# Autodesk Inventor assembly: 3_left_leg_true_final
(part 3 of 3)
Size Designation: M3 x 6
Categories: <MemberInstance><Categories><Category DisplayName="Fasteners" InternalName="e4da775c-781d-43d5-af7c-5136215cf5a6" Mnemonic="FSTN"><Category DisplayName="Bolts" InternalName="536e6df0-f778-49ac-b2f2-25c71d2aa0b2" Mnemonic="SCRW"><CategoryParameter DisplayName="Nominal Diameter Designation" InternalName="03caf894-eafd-4c09-a035-916ac084b87b" Mnemonic="nomdiadesig"/><CategoryParameter DisplayName="Nominal Length" InternalName="238ecbaf-3e6c-45dd-aa95-4068c8e0fd02" Mnemonic="nomlen"/><CategoryParameter DisplayName="Thread Designation" InternalName="586d5e89-370a-4089-914f-0110033585c7" Mnemonic="thrdesign"/><CategoryParameter DisplayName="Thread Series Designation" InternalName="87c5849c-b3a5-4c3e-9c9b-2feecef9be86" Mnemonic="thrserdsgn"/><CategoryParameter DisplayName="Nominal Diameter" InternalName="8bbe3f8e-44cf-40a9-a251-3a6edc8168d6" Mnemonic="nomdia"/><CategoryParameter DisplayName="Thread Type" InternalName="b4bbb7bc-d6aa-4c9f-a9a9-4152b9f6fe49" Mnemonic="thrtype"/><CategoryParameter DisplayName="Thread Pitch" InternalName="bb82302e-82d8-4176-8fc1-c5d7bb17d5ad" Mnemonic="pitch1"/><CategoryParameter DisplayName="Threads per Unit" InternalName="bdc6e7d2-ffd0-4d9c-a173-16b95ebb912d" Mnemonic="thrperunit1"/><CategoryParameter DisplayName="Thread Class" InternalName="ebc0d23b-2cc6-4d2a-b376-d52aae53bab6" Mnemonic="thrclss"/><Category DisplayName="Round Head" InternalName="df3578aa-538f-4805-96a8-2439eb0c3cf7" Mnemonic="RNDSCRW"><CategoryParameter DisplayName="Grip Length" InternalName="2c6ace26-543b-4217-91c4-9cdf8c3ec6f1" Mnemonic="grplen"/><CategoryParameter DisplayName="Head Height" InternalName="2d152238-84fe-49ae-94c3-3fee884c292b" Mnemonic="headh"/><CategoryParameter DisplayName="Property Class" InternalName="85496db6-1567-48ed-b0d4-aa1f03366005" Mnemonic="propclss"/><CategoryParameter DisplayName="Thread Length" InternalName="a1e5edc5-4ca7-4847-8786-65b14d35af16" Mnemonic="thrlen"/><CategoryParameter DisplayName="Shank Diameter" InternalName="c22f1a48-b8d5-43ef-ac5e-546ba91c0bd6" Mnemonic="grpdia"/><CategoryParameter DisplayName="Head Diameter" InternalName="e71ee7a1-06fd-425c-ba3b-09769885677c" Mnemonic="headdia"/></Category></Category></Category><Category DisplayName="DataType" InternalName="23b78d0f-2648-40c6-8793-ca6db495c9e8" Mnemonic="DATATYPE"><CategoryParameter DisplayName="DisplayName" InternalName="05415f3d-3907-474b-a020-eb9d644f4cf3" Mnemonic="DISPLAYNAME"/><CategoryParameter DisplayName="Standard" InternalName="0c0a119c-1e12-4c84-803f-101930972f5e" Mnemonic="STANDARD"/><CategoryParameter DisplayName="Description" InternalName="13903e3d-64b1-4950-80da-f627842ea37f" Mnemonic="DESCRIPTION"/><CategoryParameter DisplayName="Designation" InternalName="2675968c-4ce5-49e0-a4f5-552d29089031" Mnemonic="DESIGNATION"/><CategoryParameter DisplayName="Default Row" InternalName="2af9ec52-faaa-4026-b378-f9fa4afca842" Mnemonic="DEFAULTROW"/><CategoryParameter DisplayName="Folder Name" InternalName="3f06958e-8713-4116-9be7-ed6184ecc97b" Mnemonic="FOLDERNAME"/><CategoryParameter DisplayName="Revision Guid" InternalName="45a75005-10b1-4dfc-8d6d-dfe629f0b93c" Mnemonic="REVISIONGUID"/><CategoryParameter DisplayName="FileName" InternalName="8b46a4cc-9585-4fed-90c3-899f57e09a73" Mnemonic="FILENAME"/><CategoryParameter DisplayName="StdsOrg" InternalName="8f5914e1-4693-403f-8ab5-d37768198c9d" Mnemonic="STDSORG"/><CategoryParameter DisplayName="Family Version" InternalName="914462f6-6e19-4b14-ba84-155b9680b1d0" Mnemonic="FAMILYREVISION"/><CategoryParameter DisplayName="Standard Revision" InternalName="91d5a463-65c2-4fde-b823-3b7fea5e8e17" Mnemonic="STANDARDREVISION"/><CategoryParameter DisplayName="Member Revision" InternalName="a65d44b9-392f-4f4f-857b-e4b3d54996fe" Mnemonic="MEMBERREVISION"/><CategoryParameter DisplayName="ClipFormat" InternalName="bc51e27b-3422-4e78-93ef-cec197ddf230" Mnemonic="CLIPFORMAT"/><CategoryParameter DisplayName="Manufacturer" InternalName="cd6c7a72-a28a-4e50-99a9-2c7f4e13e5ad" Mnemonic="MANUFACTURER"/><CategoryParameter DisplayName="InternalName" InternalName="cf1d0246-76d9-4b4a-8305-fa0409afb5c1" Mnemonic="INTERNALNAME"/><CategoryParameter DisplayName="IsMetric" InternalName="e2385c5b-1ea4-4823-96a8-8de651266ec3" Mnemonic="ISMETRIC"/><Category DisplayName="Part" InternalName="c0e0b642-3bcb-4cc8-9e80-f96d35c4afa4" Mnemonic="PART"><CategoryParameter DisplayName="Part Number" InternalName="016b6077-bfbe-49bd-92c9-d8d59c39c941" Mnemonic="PARTNUMBER"/><CategoryParameter DisplayName="Stock Number" InternalName="4dba7c1c-e26c-444e-836c-b08b433409a8" Mnemonic="STOCKNUMBER"/><CategoryParameter DisplayName="Material Key" InternalName="5c9a8adb-dd2b-4535-b97f-0a94a95fe41f" Mnemonic="MATERIALKEY"/><CategoryParameter DisplayName="Material" InternalName="818a152a-d3c3-49ca-80ee-df7d91421b8e" Mnemonic="MATERIAL"/></Category></Category><Category DisplayName="LegacyMap" InternalName="cd87c42b-3e48-431e-b5c0-1cbeb14dfe77" Mnemonic="LEGACYMAP"><CategoryParameter DisplayName="unique DA member ID" InternalName="0918ad47-427f-4fed-ae26-24c81c58f590" Mnemonic="DACOOKIE"/><CategoryParameter DisplayName="Merge11 ID" InternalName="0ee8fb18-e2ed-4f39-96f6-1f4b5f50aa71" Mnemonic="MERGE11"/><CategoryParameter DisplayName="unique CC member ID" InternalName="5193edd4-b2b0-4ab4-9d54-de900eee34e0" Mnemonic="CCCOOKIE"/><CategoryParameter DisplayName="Split ID" InternalName="72b5c83c-be7f-45c4-ae51-9160ea6deb26" Mnemonic="SPLIT"/><CategoryParameter DisplayName="MemberID" InternalName="8e5e0294-fc51-4c8f-b3d7-003dc5ed94f6" Mnemonic="MEMBERID"/><CategoryParameter DisplayName="CatalogName" InternalName="d99d1e27-aa94-4de2-af4c-c348882a6f4f" Mnemonic="CATALOGNAME"/><CategoryParameter DisplayName="FamilyNumber" InternalName="e705e1f4-09cb-413e-91f9-551b4188271e" Mnemonic="FAMILYNUMBER"/></Category></Categories><FamilyTemplate Id="si0145"><FamilyTemplateParameters><FamilyTemplateParameter ObjectType="kUserParameterObject" ValueType="xs:double" Id="1" ObjectReferenceKey="GUL"/><FamilyTemplateParameter ObjectType="kUserParameterObject" ValueType="xs:double" Id="2" ObjectReferenceKey="SPD"/><FamilyTemplateParameter ObjectType="kUserParameterObject" ValueType="xs:double" Id="3" ObjectReferenceKey="NLG"/><FamilyTemplateParameter ObjectType="kUserParameterObject" ValueType="xs:double" Id="4" ObjectReferenceKey="TPU"/><FamilyTemplateParameter ObjectType="kUserParameterObject" ValueType="xs:double" Id="5" ObjectReferenceKey="TOA"/><FamilyTemplateParameter ObjectType="kUserParameterObject" ValueType="xs:double" Id="6" ObjectReferenceKey="GD1"/><FamilyTemplateParameter ObjectType="kUserParameterObject" ValueType="xs:double" Id="7" ObjectReferenceKey="GEL"/><FamilyTemplateParameter ObjectType="kUserParameterObject" ValueType="xs:double" Id="8" ObjectReferenceKey="SW"/><FamilyTemplateParameter ObjectType="kUserParameterObject" ValueType="xs:double" Id="9" ObjectReferenceKey="THREADDIA"/><FamilyTemplateParameter ObjectType="kUserParameterObject" ValueType="xs:double" Id="10" ObjectReferenceKey="INTI"/><FamilyTemplateParameter ObjectType="kUserParameterObject" ValueType="xs:double" Id="11" ObjectReferenceKey="BDM"/><FamilyTemplateParameter ObjectType="kUserParameterObject" ValueType="xs:double" Id="12" ObjectReferenceKey="RR"/><FamilyTemplateParameter ObjectType="kUserParameterObject" ValueType="xs:double" Id="13" ObjectReferenceKey="KOH"/><FamilyTemplateParameter ObjectType="kUserParameterObject" ValueType="xs:double" Id="14" ObjectReferenceKey="PTC"/><FamilyTemplateParameter ObjectType="kUserParameterObject" ValueType="xs:double" Id="15" ObjectReferenceKey="KOD"/><FamilyTemplateParameter ObjectType="kUserParameterObject" ValueType="xs:double" Id="16" ObjectReferenceKey="NND"/><FamilyTemplateParameter ObjectType="kUserParameterObject" ValueType="xs:double" Id="17" ObjectReferenceKey="GD"/><FamilyTemplateParameter ObjectType="kUserParameterObject" ValueType="xs:double" Id="18" ObjectReferenceKey="GAL"/><FamilyTemplateParameter ObjectType="kUserParameterObject" ValueType="xs:double" Id="19" ObjectReferenceKey="KOH1"/><FamilyTemplateParameter ObjectType="kUserParameterObject" ValueType="xs:double" Id="20" ObjectReferenceKey="E0"/><FamilyTemplateParameter ObjectType="kUserParameterObject" ValueType="xs:double" Id="132" ObjectReferenceKey="R"/><FamilyTemplateParameter ObjectType="kPropertyObject" ValueType="xs:string" Id="100" ObjectReferenceKey="{32853F0F-3444-11d1-9E93-0060B03C1CA6}" SubObjectId="52"/><FamilyTemplateParameter ObjectType="kPropertyObject" ValueType="xs:string" Id="105" ObjectReferenceKey="{32853F0F-3444-11d1-9E93-0060B03C1CA6}" SubObjectId="5"/><FamilyTemplateParameter ObjectType="kPartComponentDefinitionObject" ValueType="xs:string" Id="110" SubObjectId="Material"/><FamilyTemplateParameter ObjectType="kThreadFeatureObject" ValueType="xs:structure" Id="300" ObjectReferenceKey="1002000010000000a2070000000000008000000000000000" SubObjectId="ThreadInfo"><FamilyTemplateParameter ObjectType="" ValueType="xs:string" Id="301" SubObjectId="ThreadDesignation"/><FamilyTemplateParameter ObjectType="" ValueType="xs:string" Id="302" SubObjectId="ThreadType"/><FamilyTemplateParameter ObjectType="" ValueType="xs:string" Id="303" SubObjectId="ThreadClass"/></FamilyTemplateParameter></FamilyTemplateParameters></FamilyTemplate><CategoryParameterMap><ParamToTemplateMap><ParamToTemplate CategoryParameter="//CategoryParameter[@InternalName='05415f3d-3907-474b-a020-eb9d644f4cf3']" ConstantValue="ISO 7380-1"/><ParamToTemplate CategoryParameter="//CategoryParameter[@InternalName='cf1d0246-76d9-4b4a-8305-fa0409afb5c1']" ConstantValue="7e948a18-7d98-46c8-9f69-82be43869b08"/><ParamToTemplate CategoryParameter="//CategoryParameter[@InternalName='3f06958e-8713-4116-9be7-ed6184ecc97b']" ConstantValue="ISO 7380-1"/><ParamToTemplate CategoryParameter="//CategoryParameter[@InternalName='914462f6-6e19-4b14-ba84-155b9680b1d0']" ConstantValue="10"/><ParamToTemplate CategoryParameter="//CategoryParameter[@InternalName='bc51e27b-3422-4e78-93ef-cec197ddf230']" ConstantValue="CF_INVENTOR.STDPARTS"/><ParamToTemplate CategoryParameter="//CategoryParameter[@InternalName='e2385c5b-1ea4-4823-96a8-8de651266ec3']" ConstantValue="true"/><ParamToTemplate CategoryParameter="//CategoryParameter[@InternalName='13903e3d-64b1-4950-80da-f627842ea37f']" ConstantValue="Hexagon Socket Button Head Screw - Product grade A"/><ParamToTemplate CategoryParameter="//CategoryParameter[@InternalName='8f5914e1-4693-403f-8ab5-d37768198c9d']" ConstantValue="ISO"/><ParamToTemplate CategoryParameter="//CategoryParameter[@InternalName='0c0a119c-1e12-4c84-803f-101930972f5e']" ConstantValue="ISO 7380-1"/><ParamToTemplate CategoryParameter="//CategoryParameter[@InternalName='cd6c7a72-a28a-4e50-99a9-2c7f4e13e5ad']" TemplateParameter="104"/><ParamToTemplate CategoryParameter="//CategoryParameter[@InternalName='91d5a463-65c2-4fde-b823-3b7fea5e8e17']" ConstantValue="First edition 2011-08-01"/><ParamToTemplate CategoryParameter="//CategoryParameter[@InternalName='45a75005-10b1-4dfc-8d6d-dfe629f0b93c']" ConstantValue="28e2f25c-6dc8-4906-99e1-9c4ceb92a97a"/><ParamToTemplate CategoryParameter="//CategoryParameter[@InternalName='2af9ec52-faaa-4026-b378-f9fa4afca842']" ConstantValue="10"/><ParamToTemplate CategoryParameter="//CategoryParameter[@InternalName='d99d1e27-aa94-4de2-af4c-c348882a6f4f']" ConstantValue="ISO"/><ParamToTemplate CategoryParameter="//CategoryParameter[@InternalName='e705e1f4-09cb-413e-91f9-551b4188271e']" ConstantValue="16"/><ParamToTemplate CategoryParameter="//CategoryParameter[@InternalName='8b46a4cc-9585-4fed-90c3-899f57e09a73']" ConstantValue="ISO 7380-1 - M3 x 6"/><ParamToTemplate CategoryParameter="//CategoryParameter[@InternalName='a65d44b9-392f-4f4f-857b-e4b3d54996fe']" ConstantValue="06E58314-F7E5-4B9F-9F34-16689E4488C2"/><ParamToTemplate CategoryParameter="//CategoryParameter[@InternalName='2c6ace26-543b-4217-91c4-9cdf8c3ec6f1']" ConstantValue="1.5"/><ParamToTemplate CategoryParameter="//CategoryParameter[@InternalName='ebc0d23b-2cc6-4d2a-b376-d52aae53bab6']" ConstantValue="6g"/><ParamToTemplate CategoryParameter="//CategoryParameter[@InternalName='03caf894-eafd-4c09-a035-916ac084b87b']" ConstantValue="M3"/><ParamToTemplate CategoryParameter="//CategoryParameter[@InternalName='b4bbb7bc-d6aa-4c9f-a9a9-4152b9f6fe49']" ConstantValue="ISO Metric profile"/><ParamToTemplate CategoryParameter="//CategoryParameter[@InternalName='8e5e0294-fc51-4c8f-b3d7-003dc5ed94f6']" ConstantValue="10"/><ParamToTemplate CategoryParameter="//CategoryParameter[@InternalName='c22f1a48-b8d5-43ef-ac5e-546ba91c0bd6']" TemplateParameter="11"/><ParamToTemplate CategoryParameter="//CategoryParameter[@InternalName='2675968c-4ce5-49e0-a4f5-552d29089031']" TemplateParameter="100"/><ParamToTemplate CategoryParameter="//CategoryParameter[@InternalName='a1e5edc5-4ca7-4847-8786-65b14d35af16']" TemplateParameter="7"/><ParamToTemplate CategoryParameter="//CategoryParameter[@InternalName='e71ee7a1-06fd-425c-ba3b-09769885677c']" TemplateParameter="15"/><ParamToTemplate CategoryParameter="//CategoryParameter[@InternalName='2d152238-84fe-49ae-94c3-3fee884c292b']" TemplateParameter="13"/><ParamToTemplate CategoryParameter="//CategoryParameter[@InternalName='818a152a-d3c3-49ca-80ee-df7d91421b8e']" TemplateParameter="110"/><ParamToTemplate CategoryParameter="//CategoryParameter[@InternalName='238ecbaf-3e6c-45dd-aa95-4068c8e0fd02']" TemplateParameter="3"/><ParamToTemplate CategoryParameter="//CategoryParameter[@InternalName='8bbe3f8e-44cf-40a9-a251-3a6edc8168d6']" TemplateParameter="16"/><ParamToTemplate CategoryParameter="//CategoryParameter[@InternalName='016b6077-bfbe-49bd-92c9-d8d59c39c941']" TemplateParameter="105"/><ParamToTemplate CategoryParameter="//CategoryParameter[@InternalName='bb82302e-82d8-4176-8fc1-c5d7bb17d5ad']" TemplateParameter="14"/><ParamToTemplate CategoryParameter="//CategoryParameter[@InternalName='586d5e89-370a-4089-914f-0110033585c7']" TemplateParameter="301"/><ParamToTemplate CategoryParameter="//CategoryParameter[@InternalName='bdc6e7d2-ffd0-4d9c-a173-16b95ebb912d']" TemplateParameter="4"/></ParamToTemplateMap></CategoryParameterMap></MemberInstance>
Density: 8 g/cm^3
Appearance: Default
Sending System: Autodesk Inventor 2026
Author: chanh
## iProperties of the stored document M5 Nylon Nut.ipt
Created: 2023-01-20
Part Number: M3 Nylon Nut
Material: Stainless Steel
Description: Hexagon nuts and hexagon thin nuts
Document SubType Name: Modeling
Standard: KS B 1012
Designer: chanh
Standards Organization: KS
Language: en-US
Size Designation: M 3
Categories: <MemberInstance><Categories><Category DisplayName="Fasteners" InternalName="e4da775c-781d-43d5-af7c-5136215cf5a6" Mnemonic="FSTN"><Category DisplayName="Nuts" InternalName="e37c7a56-0470-4688-8db4-b4d75d611516" Mnemonic="NUT"><CategoryParameter DisplayName="Thread Designation" InternalName="10aefdba-3783-44b8-becc-0feae870ab73" Mnemonic="thrdesign"/><CategoryParameter DisplayName="Thread Series Designation" InternalName="17a0ae10-6923-48a9-85c7-ae9b76790e6f" Mnemonic="thrserdsgn"/><CategoryParameter DisplayName="Thread Type" InternalName="205c6614-02f1-43b1-b704-b331415a8186" Mnemonic="thrtype"/><CategoryParameter DisplayName="Nominal Diameter Designation" InternalName="39406bc0-754a-4a9f-8c64-e1bba9d40b8a" Mnemonic="nomdiadesig"/><CategoryParameter DisplayName="Height" InternalName="5579c84d-d692-41f2-8996-171d03c19b53" Mnemonic="nheig"/><CategoryParameter DisplayName="Thread Class" InternalName="9b95427d-7bb5-461a-8a3e-4650073a592b" Mnemonic="thrclss"/><CategoryParameter DisplayName="Thread Pitch" InternalName="bd2c58b1-df6d-45e3-8bf7-4a0997b15b95" Mnemonic="pitch1"/><CategoryParameter DisplayName="Nominal Diameter" InternalName="d6e3b243-37ab-4432-98ea-592d296d3a46" Mnemonic="nomdia"/><CategoryParameter DisplayName="Threads per Unit" InternalName="e2e4d09d-bc7f-4af6-8086-8693b8d97bcd" Mnemonic="thrperunit1"/><Category DisplayName="Hex" InternalName="73d9c703-2233-4460-907f-38a87f245fbb" Mnemonic="PLNUT"><CategoryParameter DisplayName="Width Across Corners" InternalName="3db1d29f-9506-4e4b-a66f-416ec1d0915f" Mnemonic="wacor"/><CategoryParameter DisplayName="Type" InternalName="4e484966-9917-44a5-bcb5-b45bf8fff7e8" Mnemonic="type"/><CategoryParameter DisplayName="Property Class" InternalName="bcb84129-2a2e-4fb9-8398-d46bb849f471" Mnemonic="propclss"/></Category></Category></Category><Category DisplayName="DataType" InternalName="23b78d0f-2648-40c6-8793-ca6db495c9e8" Mnemonic="DATATYPE"><CategoryParameter DisplayName="DisplayName" InternalName="05415f3d-3907-474b-a020-eb9d644f4cf3" Mnemonic="DISPLAYNAME"/><CategoryParameter DisplayName="Standard" InternalName="0c0a119c-1e12-4c84-803f-101930972f5e" Mnemonic="STANDARD"/><CategoryParameter DisplayName="Description" InternalName="13903e3d-64b1-4950-80da-f627842ea37f" Mnemonic="DESCRIPTION"/><CategoryParameter DisplayName="Designation" InternalName="2675968c-4ce5-49e0-a4f5-552d29089031" Mnemonic="DESIGNATION"/><CategoryParameter DisplayName="Default Row" InternalName="2af9ec52-faaa-4026-b378-f9fa4afca842" Mnemonic="DEFAULTROW"/><CategoryParameter DisplayName="Folder Name" InternalName="3f06958e-8713-4116-9be7-ed6184ecc97b" Mnemonic="FOLDERNAME"/><CategoryParameter DisplayName="Revision Guid" InternalName="45a75005-10b1-4dfc-8d6d-dfe629f0b93c" Mnemonic="REVISIONGUID"/><CategoryParameter DisplayName="FileName" InternalName="8b46a4cc-9585-4fed-90c3-899f57e09a73" Mnemonic="FILENAME"/><CategoryParameter DisplayName="StdsOrg" InternalName="8f5914e1-4693-403f-8ab5-d37768198c9d" Mnemonic="STDSORG"/><CategoryParameter DisplayName="Family Version" InternalName="914462f6-6e19-4b14-ba84-155b9680b1d0" Mnemonic="FAMILYREVISION"/><CategoryParameter DisplayName="Standard Revision" InternalName="91d5a463-65c2-4fde-b823-3b7fea5e8e17" Mnemonic="STANDARDREVISION"/><CategoryParameter DisplayName="Member Revision" InternalName="a65d44b9-392f-4f4f-857b-e4b3d54996fe" Mnemonic="MEMBERREVISION"/><CategoryParameter DisplayName="ClipFormat" InternalName="bc51e27b-3422-4e78-93ef-cec197ddf230" Mnemonic="CLIPFORMAT"/><CategoryParameter DisplayName="Manufacturer" InternalName="cd6c7a72-a28a-4e50-99a9-2c7f4e13e5ad" Mnemonic="MANUFACTURER"/><CategoryParameter DisplayName="InternalName" InternalName="cf1d0246-76d9-4b4a-8305-fa0409afb5c1" Mnemonic="INTERNALNAME"/><CategoryParameter DisplayName="IsMetric" InternalName="e2385c5b-1ea4-4823-96a8-8de651266ec3" Mnemonic="ISMETRIC"/><Category DisplayName="Part" InternalName="c0e0b642-3bcb-4cc8-9e80-f96d35c4afa4" Mnemonic="PART"><CategoryParameter DisplayName="Part Number" InternalName="016b6077-bfbe-49bd-92c9-d8d59c39c941" Mnemonic="PARTNUMBER"/><CategoryParameter DisplayName="Stock Number" InternalName="4dba7c1c-e26c-444e-836c-b08b433409a8" Mnemonic="STOCKNUMBER"/><CategoryParameter DisplayName="Material Key" InternalName="5c9a8adb-dd2b-4535-b97f-0a94a95fe41f" Mnemonic="MATERIALKEY"/><CategoryParameter DisplayName="Material" InternalName="818a152a-d3c3-49ca-80ee-df7d91421b8e" Mnemonic="MATERIAL"/></Category></Category><Category DisplayName="LegacyMap" InternalName="cd87c42b-3e48-431e-b5c0-1cbeb14dfe77" Mnemonic="LEGACYMAP"><CategoryParameter DisplayName="unique DA member ID" InternalName="0918ad47-427f-4fed-ae26-24c81c58f590" Mnemonic="DACOOKIE"/><CategoryParameter DisplayName="Merge11 ID" InternalName="0ee8fb18-e2ed-4f39-96f6-1f4b5f50aa71" Mnemonic="MERGE11"/><CategoryParameter DisplayName="unique CC member ID" InternalName="5193edd4-b2b0-4ab4-9d54-de900eee34e0" Mnemonic="CCCOOKIE"/><CategoryParameter DisplayName="Split ID" InternalName="72b5c83c-be7f-45c4-ae51-9160ea6deb26" Mnemonic="SPLIT"/><CategoryParameter DisplayName="MemberID" InternalName="8e5e0294-fc51-4c8f-b3d7-003dc5ed94f6" Mnemonic="MEMBERID"/><CategoryParameter DisplayName="CatalogName" InternalName="d99d1e27-aa94-4de2-af4c-c348882a6f4f" Mnemonic="CATALOGNAME"/><CategoryParameter DisplayName="FamilyNumber" InternalName="e705e1f4-09cb-413e-91f9-551b4188271e" Mnemonic="FAMILYNUMBER"/></Category></Categories><FamilyTemplate Id="no0141"><FamilyTemplateParameters><FamilyTemplateParameter ObjectType="kUserParameterObject" ValueType="xs:double" Id="1" ObjectReferenceKey="GUL"/><FamilyTemplateParameter ObjectType="kUserParameterObject" ValueType="xs:double" Id="2" ObjectReferenceKey="KOH"/><FamilyTemplateParameter ObjectType="kUserParameterObject" ValueType="xs:double" Id="3" ObjectReferenceKey="TPU"/><FamilyTemplateParameter ObjectType="kUserParameterObject" ValueType="xs:double" Id="4" ObjectReferenceKey="GD1"/><FamilyTemplateParameter ObjectType="kUserParameterObject" ValueType="xs:double" Id="5" ObjectReferenceKey="SW01"/><FamilyTemplateParameter ObjectType="kUserParameterObject" ValueType="xs:double" Id="6" ObjectReferenceKey="SW"/><FamilyTemplateParameter ObjectType="kUserParameterObject" ValueType="xs:double" Id="7" ObjectReferenceKey="ANG2"/><FamilyTemplateParameter ObjectType="kUserParameterObject" ValueType="xs:double" Id="8" ObjectReferenceKey="TOA"/><FamilyTemplateParameter ObjectType="kUserParameterObject" ValueType="xs:double" Id="9" ObjectReferenceKey="PTC"/><FamilyTemplateParameter ObjectType="kUserParameterObject" ValueType="xs:double" Id="10" ObjectReferenceKey="NND"/><FamilyTemplateParameter ObjectType="kUserParameterObject" ValueType="xs:double" Id="11" ObjectReferenceKey="E0"/><FamilyTemplateParameter ObjectType="kUserParameterObject" ValueType="xs:double" Id="12" ObjectReferenceKey="THREADDIA"/><FamilyTemplateParameter ObjectType="kUserParameterObject" ValueType="xs:double" Id="13" ObjectReferenceKey="GAL"/><FamilyTemplateParameter ObjectType="kPropertyObject" ValueType="xs:string" Id="100" ObjectReferenceKey="{32853F0F-3444-11d1-9E93-0060B03C1CA6}" SubObjectId="52"/><FamilyTemplateParameter ObjectType="kPropertyObject" ValueType="xs:string" Id="105" ObjectReferenceKey="{32853F0F-3444-11d1-9E93-0060B03C1CA6}" SubObjectId="5"/><FamilyTemplateParameter ObjectType="kPartComponentDefinitionObject" ValueType="xs:string" Id="110" SubObjectId="Material"/><FamilyTemplateParameter ObjectType="kThreadFeatureObject" ValueType="xs:structure" Id="300" ObjectReferenceKey="100200001000000049020000000000008000000000000000" SubObjectId="ThreadInfo"><FamilyTemplateParameter ObjectType="" ValueType="xs:string" Id="301" SubObjectId="ThreadDesignation"/><FamilyTemplateParameter ObjectType="" ValueType="xs:string" Id="302" SubObjectId="ThreadClass"/><FamilyTemplateParameter ObjectType="" ValueType="xs:string" Id="303" SubObjectId="ThreadType"/></FamilyTemplateParameter></FamilyTemplateParameters></FamilyTemplate><CategoryParameterMap><ParamToTemplateMap><ParamToTemplate CategoryParameter="//CategoryParameter[@InternalName='05415f3d-3907-474b-a020-eb9d644f4cf3']" ConstantValue="KS B 1012 Style 1 -finished - Metric"/><ParamToTemplate CategoryParameter="//CategoryParameter[@InternalName='cf1d0246-76d9-4b4a-8305-fa0409afb5c1']" ConstantValue="2b56ab5a-831b-4c97-9445-988aeee029cc"/><ParamToTemplate CategoryParameter="//CategoryParameter[@InternalName='3f06958e-8713-4116-9be7-ed6184ecc97b']" ConstantValue="KS B 1012  S1 F"/><ParamToTemplate CategoryParameter="//CategoryParameter[@InternalName='914462f6-6e19-4b14-ba84-155b9680b1d0']" ConstantValue="10"/><ParamToTemplate CategoryParameter="//CategoryParameter[@InternalName='bc51e27b-3422-4e78-93ef-cec197ddf230']" ConstantValue="CF_INVENTOR.STDPARTS"/><ParamToTemplate CategoryParameter="//CategoryParameter[@InternalName='e2385c5b-1ea4-4823-96a8-8de651266ec3']" ConstantValue="true"/><ParamToTemplate CategoryParameter="//CategoryParameter[@InternalName='13903e3d-64b1-4950-80da-f627842ea37f']" ConstantValue="Hexagon nuts and hexagon thin nuts"/><ParamToTemplate CategoryParameter="//CategoryParameter[@InternalName='8f5914e1-4693-403f-8ab5-d37768198c9d']" ConstantValue="KS"/><ParamToTemplate CategoryParameter="//CategoryParameter[@InternalName='0c0a119c-1e12-4c84-803f-101930972f5e']" ConstantValue="KS B 1012"/><ParamToTemplate CategoryParameter="//CategoryParameter[@InternalName='cd6c7a72-a28a-4e50-99a9-2c7f4e13e5ad']" TemplateParameter="104"/><ParamToTemplate CategoryParameter="//CategoryParameter[@InternalName='91d5a463-65c2-4fde-b823-3b7fea5e8e17']" TemplateParameter="103"/><ParamToTemplate CategoryParameter="//CategoryParameter[@InternalName='45a75005-10b1-4dfc-8d6d-dfe629f0b93c']" ConstantValue="9c47a41a-02a0-4062-8cd6-04c5a6321c27"/><ParamToTemplate CategoryParameter="//CategoryParameter[@InternalName='2af9ec52-faaa-4026-b378-f9fa4afca842']" ConstantValue="10"/><ParamToTemplate CategoryParameter="//CategoryParameter[@InternalName='d99d1e27-aa94-4de2-af4c-c348882a6f4f']" ConstantValue="KS"/><ParamToTemplate CategoryParameter="//CategoryParameter[@InternalName='e705e1f4-09cb-413e-91f9-551b4188271e']" ConstantValue="47"/><ParamToTemplate CategoryParameter="//CategoryParameter[@InternalName='8b46a4cc-9585-4fed-90c3-899f57e09a73']" ConstantValue="KS B 1012 - M 3(1) F"/><ParamToTemplate CategoryParameter="//CategoryParameter[@InternalName='a65d44b9-392f-4f4f-857b-e4b3d54996fe']" ConstantValue="6A642D9D-207D-4C8A-84F5-6047BF8B8DA1"/><ParamToTemplate CategoryParameter="//CategoryParameter[@InternalName='9b95427d-7bb5-461a-8a3e-4650073a592b']" ConstantValue="6H"/><ParamToTemplate CategoryParameter="//CategoryParameter[@InternalName='39406bc0-754a-4a9f-8c64-e1bba9d40b8a']" ConstantValue="M3"/><ParamToTemplate CategoryParameter="//CategoryParameter[@InternalName='205c6614-02f1-43b1-b704-b331415a8186']" ConstantValue="ISO Metric Profile"/><ParamToTemplate CategoryParameter="//CategoryParameter[@InternalName='8e5e0294-fc51-4c8f-b3d7-003dc5ed94f6']" ConstantValue="40"/><ParamToTemplate CategoryParameter="//CategoryParameter[@InternalName='2675968c-4ce5-49e0-a4f5-552d29089031']" TemplateParameter="100"/><ParamToTemplate CategoryParameter="//CategoryParameter[@InternalName='3db1d29f-9506-4e4b-a66f-416ec1d0915f']" TemplateParameter="11"/><ParamToTemplate CategoryParameter="//CategoryParameter[@InternalName='5579c84d-d692-41f2-8996-171d03c19b53']" TemplateParameter="2"/><ParamToTemplate CategoryParameter="//CategoryParameter[@InternalName='818a152a-d3c3-49ca-80ee-df7d91421b8e']" TemplateParameter="110"/><ParamToTemplate CategoryParameter="//CategoryParameter[@InternalName='d6e3b243-37ab-4432-98ea-592d296d3a46']" TemplateParameter="10"/><ParamToTemplate CategoryParameter="//CategoryParameter[@InternalName='016b6077-bfbe-49bd-92c9-d8d59c39c941']" TemplateParameter="105"/><ParamToTemplate CategoryParameter="//CategoryParameter[@InternalName='bd2c58b1-df6d-45e3-8bf7-4a0997b15b95']" TemplateParameter="9"/><ParamToTemplate CategoryParameter="//CategoryParameter[@InternalName='10aefdba-3783-44b8-becc-0feae870ab73']" TemplateParameter="301"/><ParamToTemplate CategoryParameter="//CategoryParameter[@InternalName='e2e4d09d-bc7f-4af6-8086-8693b8d97bcd']" TemplateParameter="3"/></ParamToTemplateMap></CategoryParameterMap></MemberInstance>
Density: 8 g/cm^3
Appearance: Default
Sending System: Autodesk Inventor 2026
Author: chanh
## Documents named in this file (36)
- C:\Users\User\Documents\The Maverick's Files\College 3-3\로보인 프로젝트\RHp_Humanoid_ver1\Assembly\3_left_leg_true_final.iam
- C:\Users\User\Documents\The Maverick's Files\College 3-3\로보인 프로젝트\RHp_Humanoid_ver1\Part\HTD-45H, Horn\HTD-45H\HTD-45H.iam
- C:\Users\User\Documents\The Maverick's Files\College 3-3\로보인 프로젝트\RHp_Humanoid_ver1\Part\HTD-45H, Horn\Horn\Top Horn.ipt
- C:\Users\User\Documents\The Maverick's Files\College 3-3\로보인 프로젝트\RHp_Humanoid_ver1\Part\HTD-45H, Horn\Horn\Bottom Horn.ipt
- C:\Users\User\Documents\The Maverick's Files\College 3-3\로보인 프로젝트\RHp_Humanoid_ver1\Part\Frame\Leg\Left Leg\axis_1_top_frame.ipt
- C:\Users\User\Documents\The Maverick's Files\College 3-3\로보인 프로젝트\RHp_Humanoid_ver1\Part\Frame\Leg\Left Leg\axis_3_bottom_frame.ipt
- C:\Users\User\Documents\The Maverick's Files\College 3-3\로보인 프로젝트\RHp_Humanoid_ver1\Part\Frame\Leg\Left Leg\axis_2_bottom_frame.ipt
- C:\Users\User\Documents\The Maverick's Files\College 3-3\로보인 프로젝트\RHp_Humanoid_ver1\Part\Frame\Leg\Left Leg\axis_1_supplement_frame.ipt
- C:\Users\User\Documents\The Maverick's Files\College 3-3\로보인 프로젝트\RHp_Humanoid_ver1\Part\Frame\Leg\Left Leg\axis_2_4_connector_frame_powered.ipt
- C:\Users\User\Documents\The Maverick's Files\College 3-3\로보인 프로젝트\RHp_Humanoid_ver1\Part\Frame\Leg\Left Leg\axis_2_4_connector_frame_non_powered.ipt
- C:\Users\User\Documents\The Maverick's Files\College 3-3\로보인 프로젝트\RHp_Humanoid_ver1\Part\Frame\Leg\3D_printed_part_powered.ipt
- C:\Users\User\Documents\The Maverick's Files\College 3-3\로보인 프로젝트\RHp_Humanoid_ver1\Part\Frame\Leg\3D_printed_part_non_powered.ipt
- C:\Users\User\Documents\The Maverick's Files\College 3-3\로보인 프로젝트\RHp_Humanoid_ver1\Part\Frame\Leg\Left Leg\axis_4_5_connector_frame_powered.ipt
- C:\Users\User\Documents\The Maverick's Files\College 3-3\로보인 프로젝트\RHp_Humanoid_ver1\Part\Frame\Leg\Left Leg\axis_4_5_connector_frame_non_powered.ipt
- C:\Users\User\Documents\The Maverick's Files\College 3-3\로보인 프로젝트\RHp_Humanoid_ver1\Part\Frame\Leg\Left Leg\axis_5_top_frame.ipt
- C:\Users\User\Documents\The Maverick's Files\College 3-3\로보인 프로젝트\RHp_Humanoid_ver1\Part\Frame\Leg\Left Leg\axis_6_top_frame.ipt
- C:\Users\User\Documents\The Maverick's Files\College 3-3\로보인 프로젝트\RHp_Humanoid_ver1\Part\Frame\Leg\Left Leg\axis_6_bottom_frame(top).ipt
- C:\Users\User\Documents\The Maverick's Files\College 3-3\로보인 프로젝트\RHp_Humanoid_ver1\Part\Frame\Leg\Left Leg\axis_6_bottom_frame(bottom).ipt
- C:\Users\User\Documents\The Maverick's Files\College 3-3\로보인 프로젝트\RHp_Humanoid_ver1\Part\Frame\Leg\Left Leg\axis_6_supplement_frame.ipt
- **C:\Users\User\Documents\The Maverick's Files\College 3-3\로보인 프로젝트\RHp_Humanoid_ver1\Assembly\3_left_leg_true_final.iam*LocalDocs*xAaaaqobaAaaaaaaaAaaaaizvZc*M5x10 Bolt.ipt
- **C:\Users\User\Documents\The Maverick's Files\College 3-3\로보인 프로젝트\RHp_Humanoid_ver1\Assembly\3_left_leg_true_final.iam*LocalDocs*xAaaaqybaAaaaaaaaAaaaaqveUh*M5 Nylon Nut.ipt
- **C:\Users\User\Documents\The Maverick's Files\College 3-3\로보인 프로젝트\RHp_Humanoid_ver1\Assembly\3_left_leg_true_final.iam*LocalDocs*xAaaaqsdaAaaaaaaaAaaaqxjeWe*M3x6 Bolt.ipt
- C:\Users\User\Documents\The Maverick's Files\College 3-3\로보인 프로젝트\RHp_Humanoid_ver1\Part\Bolt, Bearing, Nut, Washer\볼트, 너트\볼트, 너트\M3 Nut.ipt
- **C:\Users\User\Documents\The Maverick's Files\College 3-3\로보인 프로젝트\RHp_Humanoid_ver1\Assembly\3_left_leg_true_final.iam*LocalDocs*xAaaaqwcaAaaaaaaaAaaaqydaXe*M2x6 Bolt.ipt
- **C:\Users\User\Documents\The Maverick's Files\College 3-3\로보인 프로젝트\RHp_Humanoid_ver1\Assembly\3_left_leg_true_final.iam*LocalDocs*xAaaaqeaaAaaaaaaaAaaaqigk3b*M2x4 Bolt.ipt
- **C:\Users\User\Documents\The Maverick's Files\College 3-3\로보인 프로젝트\RHp_Humanoid_ver1\Assembly\3_left_leg_true_final.iam*LocalDocs*xAaaaalcaAaaaaaaaAaaaarhpKa*M2x12 Bolt.ipt
- **C:\Users\User\Documents\The Maverick's Files\College 3-3\로보인 프로젝트\RHp_Humanoid_ver1\Assembly\3_left_leg_true_final.iam*LocalDocs*xAaaaatdaAaaaaaaaAaaaajgoFe*M2x8접시.ipt
- **C:\Users\User\Documents\The Maverick's Files\College 3-3\로보인 프로젝트\RHp_Humanoid_ver1\Assembly\3_left_leg_true_final.iam*LocalDocs*xAaaaq1aaAaaaaaaaAaaaqjp0Ad*M2x45 Bolt.ipt
- C:\Users\User\Documents\The Maverick's Files\College 3-3\로보인 프로젝트\RHp_Humanoid_ver1\Part\Bolt, Bearing, Nut, Washer\볼트, 너트\볼트, 너트\M5x10 Bolt.ipt
- C:\Users\User\Documents\The Maverick's Files\College 3-3\로보인 프로젝트\RHp_Humanoid_ver1\Part\Bolt, Bearing, Nut, Washer\볼트, 너트\볼트, 너트\M5 Nylon Nut.ipt
- C:\Users\User\Documents\The Maverick's Files\College 3-3\로보인 프로젝트\RHp_Humanoid_ver1\Part\Bolt, Bearing, Nut, Washer\볼트, 너트\볼트, 너트\M3x6 Bolt.ipt
- C:\Users\User\Documents\The Maverick's Files\College 3-3\로보인 프로젝트\RHp_Humanoid_ver1\Part\Bolt, Bearing, Nut, Washer\볼트, 너트\볼트, 너트\M2x6 Bolt.ipt
- C:\Users\User\Documents\The Maverick's Files\College 3-3\로보인 프로젝트\RHp_Humanoid_ver1\Part\Bolt, Bearing, Nut, Washer\볼트, 너트\볼트, 너트\M2x4 Bolt.ipt
- C:\Users\User\Documents\The Maverick's Files\College 3-3\로보인 프로젝트\RHp_Humanoid_ver1\Part\Bolt, Bearing, Nut, Washer\볼트, 너트\볼트, 너트\M2x12 Bolt.ipt
- C:\Users\User\Documents\The Maverick's Files\College 3-3\로보인 프로젝트\RHp_Humanoid_ver1\Part\Bolt, Bearing, Nut, Washer\볼트, 너트\볼트, 너트\M2x8접시.ipt
- C:\Users\User\Documents\The Maverick's Files\College 3-3\로보인 프로젝트\RHp_Humanoid_ver1\Part\Bolt, Bearing, Nut, Washer\볼트, 너트\볼트, 너트\M2x45 Bolt.ipt
## Components (128 placed, 27 different names)
1. HTD-45H:1 [sub-assembly] — Rotational:1
2. Top Horn:1 — Rotational:1, Rigid:1
3. axis_1_top_frame:1 — Rigid:1, Rigid:2, Rigid:5, Rigid:29
4. axis_1_supplement_frame:1 — Rigid:5, Rigid:28, Rigid:83, Rigid:80, Rigid:81, Rigid:82, Rigid:84, Rigid:85, Rigid:86, Rigid:87
5. HTD-45H:3 [sub-assembly] — Rotational:3, Rigid:25
6. Top Horn:3 — Rotational:3, Rigid:7
7. Bottom Horn:3 — Rigid:8
8. axis_2_bottom_frame:1 — Rigid:25, Rigid:27, Rigid:36, Rigid:37, Rigid:38, Rigid:39, Rigid:62, Rigid:63, Rigid:64, Rigid:65, Rigid:66, Rigid:67, Rigid:68, Rigid:69, Rigid:70
9. axis_2_4_connector_frame_powered:1 — Rigid:7, Rigid:23, Rigid:96, Rigid:97, Rigid:98, Rigid:99, Rigid:113, Rigid:114, Rigid:115, Rigid:125, Rigid:126
10. axis_2_4_connector_frame_non_powered:1 — Rigid:8, Rigid:24, Rigid:108, Rigid:109, Rigid:110, Rigid:111, Rigid:116, Rigid:117, Rigid:118
11. HTD-45H:2 [sub-assembly] — Rotational:2, Rigid:26
12. Top Horn:2 — Rotational:2, Rigid:2
13. axis_3_bottom_frame:1 — Rigid:26, Rigid:27, Rigid:44, Rigid:45, Rigid:46, Rigid:47, Rigid:71, Rigid:72, Rigid:73, Rigid:74, Rigid:75
14. HTD-45H:4 [sub-assembly] — Rotational:5, Rigid:11, Rigid:21, Rotational:113
15. Top Horn:4 — Rotational:5, Rigid:12
16. Bottom Horn:4 — Rigid:13, Rotational:113
17. 3D_printed_part_powered:1 — Rigid:11, Rigid:23
18. 3D_printed_part_non_powered:1 — Rigid:21, Rigid:24
19. axis_4_5_connector_frame_powered:1 — Rigid:12, Rigid:88, Rigid:89, Rigid:90, Rigid:91, Rigid:92, Rigid:93, Rigid:94, Rigid:95, Rigid:112
20. axis_4_5_connector_frame_non_powered:1 — Rigid:13, Rigid:22, Rigid:100, Rigid:101, Rigid:102, Rigid:103, Rigid:104, Rigid:105, Rigid:106, Rigid:107
21. HTD-45H:5 [sub-assembly] — Rotational:7, Rotational:8, Rigid:14
22. Top Horn:5 — Rotational:7, Rigid:112
23. Bottom Horn:5 — Rotational:8, Rigid:22
24. axis_5_top_frame:1 — Rigid:14, Rigid:17, Rigid:40, Rigid:41, Rigid:42, Rigid:43, Rigid:48, Rigid:49, Rigid:50, Rigid:51, Rigid:52, Rigid:53, Rigid:54, Rigid:55, Rigid:56
25. HTD-45H:6 [sub-assembly] — Rigid:16, Rotational:9
26. Top Horn:6 — Rotational:9, Rigid:19
27. axis_6_top_frame:1 — Rigid:16, Rigid:17, Rigid:32, Rigid:33, Rigid:34, Rigid:35, Rigid:57, Rigid:58, Rigid:59, Rigid:60, Rigid:61
28. axis_6_supplement_frame:1 — Rigid:18, Rigid:30, Rigid:76, Rigid:77, Rigid:78, Rigid:79
29. axis_6_bottom_frame(top):1 — Rigid:18, Rigid:19, Rigid:20, Rigid:31
30. axis_6_bottom_frame(bottom):1 — Rigid:20, Rigid:119, Rigid:120, Rigid:121, Rigid:122, Rigid:123, Rigid:124
31. M2x4 Bolt:1 — Rigid:88
32. M2x4 Bolt:2 — Rigid:89
33. M2x4 Bolt:3 — Rigid:90
34. M2x4 Bolt:4 — Rigid:91
35. M2x4 Bolt:5 — Rigid:92
36. M2x4 Bolt:6 — Rigid:93
37. M2x4 Bolt:7 — Rigid:94
38. M2x4 Bolt:8 — Rigid:95
39. M2x4 Bolt:9 — Rigid:96
40. M2x4 Bolt:10 — Rigid:97
41. M2x4 Bolt:11 — Rigid:98
42. M2x4 Bolt:12 — Rigid:99
43. M2x4 Bolt:13 — Rigid:100
44. M2x4 Bolt:14 — Rigid:101
45. M2x4 Bolt:15 — Rigid:102
46. M2x4 Bolt:16 — Rigid:103
47. M2x4 Bolt:17 — Rigid:104
48. M2x4 Bolt:18 — Rigid:105
49. M2x4 Bolt:19 — Rigid:106
50. M2x4 Bolt:20 — Rigid:107
51. M2x4 Bolt:21 — Rigid:108
52. M2x4 Bolt:22 — Rigid:109
53. M2x4 Bolt:23 — Rigid:110
54. M2x4 Bolt:24 — Rigid:111
55. M2x6 Bolt:1 — Rigid:48
56. M2x6 Bolt:2 — Rigid:49
57. M2x6 Bolt:3 — Rigid:50
58. M2x6 Bolt:4 — Rigid:51
59. M2x6 Bolt:5 — Rigid:52
60. M2x6 Bolt:6 — Rigid:53
61. M2x6 Bolt:7 — Rigid:54
62. M2x6 Bolt:8 — Rigid:55
63. M2x6 Bolt:9 — Rigid:56
64. M2x6 Bolt:10 — Rigid:57
65. M2x6 Bolt:11 — Rigid:58
66. M2x6 Bolt:12 — Rigid:59
67. M2x6 Bolt:13 — Rigid:60
68. M2x6 Bolt:14 — Rigid:61
69. M2x6 Bolt:15 — Rigid:62
70. M2x6 Bolt:16 — Rigid:63
71. M2x6 Bolt:17 — Rigid:64
72. M2x6 Bolt:18 — Rigid:65
73. M2x6 Bolt:19 — Rigid:66
74. M2x6 Bolt:20 — Rigid:67
75. M2x6 Bolt:21 — Rigid:68
76. M2x6 Bolt:22 — Rigid:69
77. M2x6 Bolt:23 — Rigid:70
78. M2x6 Bolt:24 — Rigid:71
79. M2x6 Bolt:25 — Rigid:72
80. M2x6 Bolt:26 — Rigid:73
81. M2x6 Bolt:27 — Rigid:74
82. M2x6 Bolt:28 — Rigid:75
83. M2x6 Bolt:29 — Rigid:76
84. M2x6 Bolt:30 — Rigid:77
85. M2x6 Bolt:31 — Rigid:78
86. M2x6 Bolt:32 — Rigid:79
87. M2x6 Bolt:33 — Rigid:83
88. M2x6 Bolt:34 — Rigid:80
89. M2x6 Bolt:35 — Rigid:81
90. M2x6 Bolt:36 — Rigid:82
91. M2x6 Bolt:37 — Rigid:84
92. M2x6 Bolt:38 — Rigid:85
93. M2x6 Bolt:39 — Rigid:86
94. M2x6 Bolt:40 — Rigid:87
95. M2x8접시:1 — Rigid:119
96. M2x8접시:2 — Rigid:120
97. M2x8접시:3 — Rigid:121
98. M2x8접시:4 — Rigid:122
99. M2x8접시:5 — Rigid:123
100. M2x8접시:6 — Rigid:124
101. M2x12 Bolt:1 — Rigid:113
102. M2x12 Bolt:2 — Rigid:114
103. M2x12 Bolt:3 — Rigid:115
104. M2x12 Bolt:4 — Rigid:116
105. M2x12 Bolt:5 — Rigid:117
106. M2x12 Bolt:6 — Rigid:118
107. M2x45 Bolt:1 — Rigid:125
108. M2x45 Bolt:2 — Rigid:126
109. M3x6 Bolt:1 — Rigid:33
110. M3x6 Bolt:2 — Rigid:32
111. M3x6 Bolt:3 — Rigid:34
112. M3x6 Bolt:4 — Rigid:35
113. M3x6 Bolt:5 — Rigid:36
114. M3x6 Bolt:6 — Rigid:37
115. M3x6 Bolt:7 — Rigid:38
116. M3x6 Bolt:8 — Rigid:39
117. M3 Nut:1 — Rigid:40
118. M3 Nut:2 — Rigid:41
119. M3 Nut:3 — Rigid:42
120. M3 Nut:4 — Rigid:43
121. M3 Nut:5 — Rigid:44
122. M3 Nut:6 — Rigid:45
123. M3 Nut:7 — Rigid:46
124. M3 Nut:8 — Rigid:47
125. M5x10 Bolt:1 — Rigid:30
126. M5x10 Bolt:4 — Rigid:28
127. M5 Nylon Nut:1 — Rigid:29
128. M5 Nylon Nut:2 — Rigid:31
## Relationships (128: WeldJoint 120, RevoluteJoint 8)
- Rotational:1 [RevoluteJoint]: HTD-45H:1 ↔ Top Horn:1
- Rigid:1 [WeldJoint]: Top Horn:1 ↔ axis_1_top_frame:1
- Rotational:2 [RevoluteJoint]: HTD-45H:2 ↔ Top Horn:2
- Rigid:2 [WeldJoint]: axis_1_top_frame:1 ↔ Top Horn:2
- Rotational:3 [RevoluteJoint]: HTD-45H:3 ↔ Top Horn:3
- Rigid:5 [WeldJoint]: axis_1_top_frame:1 ↔ axis_1_supplement_frame:1
- Rigid:7 [WeldJoint]: Top Horn:3 ↔ axis_2_4_connector_frame_powered:1
- Rigid:8 [WeldJoint]: Bottom Horn:3 ↔ axis_2_4_connector_frame_non_powered:1
- Rotational:5 [RevoluteJoint]: HTD-45H:4 ↔ Top Horn:4
- Rigid:11 [WeldJoint]: HTD-45H:4 ↔ 3D_printed_part_powered:1
- Rigid:12 [WeldJoint]: Top Horn:4 ↔ axis_4_5_connector_frame_powered:1
- Rigid:13 [WeldJoint]: Bottom Horn:4 ↔ axis_4_5_connector_frame_non_powered:1
- Rotational:7 [RevoluteJoint]: HTD-45H:5 ↔ Top Horn:5
- Rotational:8 [RevoluteJoint]: HTD-45H:5 ↔ Bottom Horn:5
- Rigid:14 [WeldJoint]: HTD-45H:5 ↔ axis_5_top_frame:1
- Rigid:16 [WeldJoint]: HTD-45H:6 ↔ axis_6_top_frame:1
- Rotational:9 [RevoluteJoint]: HTD-45H:6 ↔ Top Horn:6
- Rigid:17 [WeldJoint]: axis_5_top_frame:1 ↔ axis_6_top_frame:1
- Rigid:18 [WeldJoint]: axis_6_supplement_frame:1 ↔ axis_6_bottom_frame(top):1
- Rigid:19 [WeldJoint]: Top Horn:6 ↔ axis_6_bottom_frame(top):1
- Rigid:20 [WeldJoint]: axis_6_bottom_frame(top):1 ↔ axis_6_bottom_frame(bottom):1
- Rigid:21 [WeldJoint]: HTD-45H:4 ↔ 3D_printed_part_non_powered:1
- Rigid:22 [WeldJoint]: axis_4_5_connector_frame_non_powered:1 ↔ Bottom Horn:5
- Rigid:23 [WeldJoint]: axis_2_4_connector_frame_powered:1 ↔ 3D_printed_part_powered:1
- Rigid:24 [WeldJoint]: axis_2_4_connector_frame_non_powered:1 ↔ 3D_printed_part_non_powered:1
- Rigid:25 [WeldJoint]: HTD-45H:3 ↔ axis_2_bottom_frame:1
- Rigid:26 [WeldJoint]: HTD-45H:2 ↔ axis_3_bottom_frame:1
- Rigid:27 [WeldJoint]: axis_2_bottom_frame:1 ↔ axis_3_bottom_frame:1
- Rigid:28 [WeldJoint]: axis_1_supplement_frame:1 ↔ M5x10 Bolt:4
- Rigid:29 [WeldJoint]: axis_1_top_frame:1 ↔ M5 Nylon Nut:1
- Rigid:30 [WeldJoint]: axis_6_supplement_frame:1 ↔ M5x10 Bolt:1
- Rigid:31 [WeldJoint]: axis_6_bottom_frame(top):1 ↔ M5 Nylon Nut:2
- Rigid:32 [WeldJoint]: axis_6_top_frame:1 ↔ M3x6 Bolt:2
- Rigid:33 [WeldJoint]: axis_6_top_frame:1 ↔ M3x6 Bolt:1
- Rigid:34 [WeldJoint]: axis_6_top_frame:1 ↔ M3x6 Bolt:3
- Rigid:35 [WeldJoint]: axis_6_top_frame:1 ↔ M3x6 Bolt:4
- Rigid:36 [WeldJoint]: axis_2_bottom_frame:1 ↔ M3x6 Bolt:5
- Rigid:37 [WeldJoint]: axis_2_bottom_frame:1 ↔ M3x6 Bolt:6
- Rigid:38 [WeldJoint]: axis_2_bottom_frame:1 ↔ M3x6 Bolt:7
- Rigid:39 [WeldJoint]: axis_2_bottom_frame:1 ↔ M3x6 Bolt:8
- Rigid:40 [WeldJoint]: axis_5_top_frame:1 ↔ M3 Nut:1
- Rigid:41 [WeldJoint]: axis_5_top_frame:1 ↔ M3 Nut:2
- Rigid:42 [WeldJoint]: axis_5_top_frame:1 ↔ M3 Nut:3
- Rigid:43 [WeldJoint]: axis_5_top_frame:1 ↔ M3 Nut:4
- Rigid:44 [WeldJoint]: axis_3_bottom_frame:1 ↔ M3 Nut:5
- Rigid:45 [WeldJoint]: axis_3_bottom_frame:1 ↔ M3 Nut:6
- Rigid:46 [WeldJoint]: axis_3_bottom_frame:1 ↔ M3 Nut:7
- Rigid:47 [WeldJoint]: axis_3_bottom_frame:1 ↔ M3 Nut:8
- Rigid:48 [WeldJoint]: axis_5_top_frame:1 ↔ M2x6 Bolt:1
- Rigid:49 [WeldJoint]: axis_5_top_frame:1 ↔ M2x6 Bolt:2
- Rigid:50 [WeldJoint]: axis_5_top_frame:1 ↔ M2x6 Bolt:3
- Rigid:51 [WeldJoint]: axis_5_top_frame:1 ↔ M2x6 Bolt:4
- Rigid:52 [WeldJoint]: axis_5_top_frame:1 ↔ M2x6 Bolt:5
- Rigid:53 [WeldJoint]: axis_5_top_frame:1 ↔ M2x6 Bolt:6
- Rigid:54 [WeldJoint]: axis_5_top_frame:1 ↔ M2x6 Bolt:7
- Rigid:55 [WeldJoint]: axis_5_top_frame:1 ↔ M2x6 Bolt:8
- Rigid:56 [WeldJoint]: axis_5_top_frame:1 ↔ M2x6 Bolt:9
- Rigid:57 [WeldJoint]: axis_6_top_frame:1 ↔ M2x6 Bolt:10
- Rigid:58 [WeldJoint]: axis_6_top_frame:1 ↔ M2x6 Bolt:11
- Rigid:59 [WeldJoint]: axis_6_top_frame:1 ↔ M2x6 Bolt:12
- Rigid:60 [WeldJoint]: axis_6_top_frame:1 ↔ M2x6 Bolt:13
- Rigid:61 [WeldJoint]: axis_6_top_frame:1 ↔ M2x6 Bolt:14
- Rigid:62 [WeldJoint]: axis_2_bottom_frame:1 ↔ M2x6 Bolt:15
- Rigid:63 [WeldJoint]: axis_2_bottom_frame:1 ↔ M2x6 Bolt:16
- Rigid:64 [WeldJoint]: axis_2_bottom_frame:1 ↔ M2x6 Bolt:17
- Rigid:65 [WeldJoint]: axis_2_bottom_frame:1 ↔ M2x6 Bolt:18
- Rigid:66 [WeldJoint]: axis_2_bottom_frame:1 ↔ M2x6 Bolt:19
- Rigid:67 [WeldJoint]: axis_2_bottom_frame:1 ↔ M2x6 Bolt:20
- Rigid:68 [WeldJoint]: axis_2_bottom_frame:1 ↔ M2x6 Bolt:21
- Rigid:69 [WeldJoint]: axis_2_bottom_frame:1 ↔ M2x6 Bolt:22
- Rigid:70 [WeldJoint]: axis_2_bottom_frame:1 ↔ M2x6 Bolt:23
- Rigid:71 [WeldJoint]: axis_3_bottom_frame:1 ↔ M2x6 Bolt:24
- Rigid:72 [WeldJoint]: axis_3_bottom_frame:1 ↔ M2x6 Bolt:25
- Rigid:73 [WeldJoint]: axis_3_bottom_frame:1 ↔ M2x6 Bolt:26
- Rigid:74 [WeldJoint]: axis_3_bottom_frame:1 ↔ M2x6 Bolt:27
- Rigid:75 [WeldJoint]: axis_3_bottom_frame:1 ↔ M2x6 Bolt:28
- Rigid:76 [WeldJoint]: axis_6_supplement_frame:1 ↔ M2x6 Bolt:29
- Rigid:77 [WeldJoint]: axis_6_supplement_frame:1 ↔ M2x6 Bolt:30
- Rigid:78 [WeldJoint]: axis_6_supplement_frame:1 ↔ M2x6 Bolt:31
- Rigid:79 [WeldJoint]: axis_6_supplement_frame:1 ↔ M2x6 Bolt:32
- Rigid:83 [WeldJoint]: axis_1_supplement_frame:1 ↔ M2x6 Bolt:33
- Rigid:80 [WeldJoint]: axis_1_supplement_frame:1 ↔ M2x6 Bolt:34
- Rigid:81 [WeldJoint]: axis_1_supplement_frame:1 ↔ M2x6 Bolt:35
- Rigid:82 [WeldJoint]: axis_1_supplement_frame:1 ↔ M2x6 Bolt:36
- Rigid:84 [WeldJoint]: axis_1_supplement_frame:1 ↔ M2x6 Bolt:37
- Rigid:85 [WeldJoint]: axis_1_supplement_frame:1 ↔ M2x6 Bolt:38
- Rigid:86 [WeldJoint]: axis_1_supplement_frame:1 ↔ M2x6 Bolt:39
- Rigid:87 [WeldJoint]: axis_1_supplement_frame:1 ↔ M2x6 Bolt:40
- Rigid:88 [WeldJoint]: axis_4_5_connector_frame_powered:1 ↔ M2x4 Bolt:1
- Rigid:89 [WeldJoint]: axis_4_5_connector_frame_powered:1 ↔ M2x4 Bolt:2
- Rigid:90 [WeldJoint]: axis_4_5_connector_frame_powered:1 ↔ M2x4 Bolt:3
- Rigid:91 [WeldJoint]: axis_4_5_connector_frame_powered:1 ↔ M2x4 Bolt:4
- Rigid:92 [WeldJoint]: axis_4_5_connector_frame_powered:1 ↔ M2x4 Bolt:5
- Rigid:93 [WeldJoint]: axis_4_5_connector_frame_powered:1 ↔ M2x4 Bolt:6
- Rigid:94 [WeldJoint]: axis_4_5_connector_frame_powered:1 ↔ M2x4 Bolt:7
- Rigid:95 [WeldJoint]: axis_4_5_connector_frame_powered:1 ↔ M2x4 Bolt:8
- Rigid:96 [WeldJoint]: axis_2_4_connector_frame_powered:1 ↔ M2x4 Bolt:9
- Rigid:97 [WeldJoint]: axis_2_4_connector_frame_powered:1 ↔ M2x4 Bolt:10
- Rigid:98 [WeldJoint]: axis_2_4_connector_frame_powered:1 ↔ M2x4 Bolt:11
- Rigid:99 [WeldJoint]: axis_2_4_connector_frame_powered:1 ↔ M2x4 Bolt:12
- Rigid:100 [WeldJoint]: axis_4_5_connector_frame_non_powered:1 ↔ M2x4 Bolt:13
- Rigid:101 [WeldJoint]: axis_4_5_connector_frame_non_powered:1 ↔ M2x4 Bolt:14
- Rigid:102 [WeldJoint]: axis_4_5_connector_frame_non_powered:1 ↔ M2x4 Bolt:15
- Rigid:103 [WeldJoint]: axis_4_5_connector_frame_non_powered:1 ↔ M2x4 Bolt:16
- Rigid:104 [WeldJoint]: axis_4_5_connector_frame_non_powered:1 ↔ M2x4 Bolt:17
- Rigid:105 [WeldJoint]: axis_4_5_connector_frame_non_powered:1 ↔ M2x4 Bolt:18
- Rigid:106 [WeldJoint]: axis_4_5_connector_frame_non_powered:1 ↔ M2x4 Bolt:19
- Rigid:107 [WeldJoint]: axis_4_5_connector_frame_non_powered:1 ↔ M2x4 Bolt:20
- Rigid:108 [WeldJoint]: axis_2_4_connector_frame_non_powered:1 ↔ M2x4 Bolt:21
- Rigid:109 [WeldJoint]: axis_2_4_connector_frame_non_powered:1 ↔ M2x4 Bolt:22
- Rigid:110 [WeldJoint]: axis_2_4_connector_frame_non_powered:1 ↔ M2x4 Bolt:23
- Rigid:111 [WeldJoint]: axis_2_4_connector_frame_non_powered:1 ↔ M2x4 Bolt:24
- Rotational:113 [RevoluteJoint]: HTD-45H:4 ↔ Bottom Horn:4
- Rigid:112 [WeldJoint]: axis_4_5_connector_frame_powered:1 ↔ Top Horn:5
- Rigid:113 [WeldJoint]: axis_2_4_connector_frame_powered:1 ↔ M2x12 Bolt:1
- Rigid:114 [WeldJoint]: axis_2_4_connector_frame_powered:1 ↔ M2x12 Bolt:2
- Rigid:115 [WeldJoint]: axis_2_4_connector_frame_powered:1 ↔ M2x12 Bolt:3
- Rigid:116 [WeldJoint]: axis_2_4_connector_frame_non_powered:1 ↔ M2x12 Bolt:4
- Rigid:117 [WeldJoint]: axis_2_4_connector_frame_non_powered:1 ↔ M2x12 Bolt:5
- Rigid:118 [WeldJoint]: axis_2_4_connector_frame_non_powered:1 ↔ M2x12 Bolt:6
- Rigid:119 [WeldJoint]: axis_6_bottom_frame(bottom):1 ↔ M2x8접시:1
- Rigid:120 [WeldJoint]: axis_6_bottom_frame(bottom):1 ↔ M2x8접시:2
- Rigid:121 [WeldJoint]: axis_6_bottom_frame(bottom):1 ↔ M2x8접시:3
- Rigid:122 [WeldJoint]: axis_6_bottom_frame(bottom):1 ↔ M2x8접시:4
- Rigid:123 [WeldJoint]: axis_6_bottom_frame(bottom):1 ↔ M2x8접시:5
- Rigid:124 [WeldJoint]: axis_6_bottom_frame(bottom):1 ↔ M2x8접시:6
- Rigid:125 [WeldJoint]: axis_2_4_connector_frame_powered:1 ↔ M2x45 Bolt:1
- Rigid:126 [WeldJoint]: axis_2_4_connector_frame_powered:1 ↔ M2x45 Bolt:2
